# Autodesk Inventor assembly: WheelAssembly
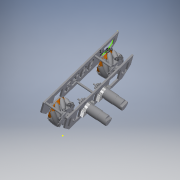
[picture p0: Inventor's stored thumbnail of the model, 180x180]
Saved by Autodesk Inventor 2017 (Build 210142000, 142)
## iProperties
Created: 2016-09-10
Part Number: WheelAssembly
Document SubType Name: Assembly
Designer: RoboticsUser
Author: RoboticsUser
## Documents named in this file (13)
- C:\Robotics\CAD\2016-17_CAD\Sub-Assemblies\MechanumNexus'AdaptorLeft - Copy.iam
- C:\Robotics\CAD\COTSParts\Actobotics\545 parts\545556.ipt
- C:\Robotics\CAD\COTSParts\Actobotics\615 parts\615102.ipt
- C:\Robotics\CAD\COTSParts\Actobotics\634 parts\634080.ipt
- C:\Robotics\CAD\COTSParts\Motors\Andymark 2964  NeveRest 40 Motor.ipt
- C:\Robotics\CAD\COTSParts\Tetrix\tetrix-motor-mounts-1.snapshot.1\Tetrex 2pc motor mount.ipt
- C:\Robotics\CAD\COTSParts\Actobotics\545 parts\545456.ipt
- C:\Robotics\CAD\COTSParts\Wheels\AndyMark Mecanum Wheels\100mm Aluminum Mecanum wheels.ipt
- C:\Robotics\CAD\2016-17_CAD\DriveTrain\DrainTrainPlate2.0LeftOutside.iam
- C:\Robotics\CAD\2016-17_CAD\DriveTrain\DriveTrainPlate2.0LeftInside.ipt
- C:\Robotics\CAD\COTSParts\Actobotics\535 parts\535198.ipt
- C:\Robotics\CAD\COTSParts\Actobotics\collar.ipt
- C:\Robotics\CAD\2016-17_CAD\DriveTrain\drive train standoff.ipt
## Components (35 placed, 12 different names)
1. 545556:2 — Mate:34, Mate:35, Mate:36, Mate:43
2. 615102:4 — Mate:62, Flush:6, Mate:65
3. 634080:2 — Mate:18, Flush:2, Mate:20, Mate:22, Mate:25, Mate:29, Mate:30, Mate:33, Mate:35, Mate:44, Mate:46, Mate:48
4. 545556:6 — Mate:8, Mate:17, Mate:27
5. 634080:3 — Mate:1, Mate:2, Mate:4, Mate:5, Mate:8, Mate:10, Mate:12, Flush:1, Mate:13, Mate:15, Mate:40, Mate:42, Mate:47
6. Andymark 2964  NeveRest 40 Motor:2 — Flush:3, Mate:59, Mate:62, Mate:66
7. 545556:8 — Mate:65, Mate:66
8. 545556:9 — Mate:63, Mate:64
9. Tetrex 2pc motor mount:1 — Mate:56, Mate:57, Mate:59
10. Tetrex 2pc motor mount:2 — Mate:58, Insert:1, Mate:60
11. 545456:1 — Mate:32, Mate:33, Mate:34, Mate:37
12. 545456:3 — Mate:9, Mate:10, Mate:27
13. 615102:6 — Flush:5, Mate:61, Mate:63
14. 615102:7 — Mate:36, Mate:37, Flush:5
15. 100mm Aluminum Mecanum wheels:1 — Mate:1, Mate:3, Mate:9
16. 100mm Aluminum Mecanum wheels:2 — Mate:30, Mate:31, Mate:32
17. 545456:4 — Mate:28, Mate:29, Mate:31
18. 545456:5 — Mate:2, Mate:3, Mate:7, Mate:38
19. 545556:13 — Mate:23, Mate:24, Mate:25, Mate:28
20. 545556:12 — Mate:4, Mate:38, Mate:39
21. DriveTrainPlate2.0LeftInside:1 — Mate:47, Mate:48, Mate:49, Mate:56, Mate:57, Mate:58, Insert:1, Flush:3, Flush:4
22. 615102:8 — Mate:5, Mate:7, Flush:6
23. 535198:2 — Mate:41, Mate:42
24. 535198:3 — Mate:45, Mate:46, Mate:49
25. 535198:4 — Mate:19, Mate:20, Mate:21
26. 535198:5 — Mate:14, Mate:15, Mate:16
27. collar:1 — Mate:21, Mate:22, Mate:23, Mate:24
28. collar:2 — Mate:13, Mate:16, Mate:17
29. Andymark 2964  NeveRest 40 Motor:3 — Flush:4, Mate:60, Mate:61, Mate:64
30. collar:3 — Mate:43, Mate:44, Mate:45
31. collar:4 — Mate:39, Mate:40, Mate:41
32. drive train standoff:1 — Mate:50, Mate:51
33. drive train standoff:2 — Mate:54, Mate:55
34. drive train standoff:3 — Mate:52, Mate:53
35. DrainTrainPlate2.0LeftOutside:1 [sub-assembly] — Mate:12, Flush:1, Mate:14, Mate:18, Flush:2, Mate:19, Mate:50, Mate:51, Mate:52, Mate:53, Mate:54, Mate:55
## Relationships (70: Mate 63, Flush 6, Insert 1)
- Mate:1: 634080:3 ↔ 100mm Aluminum Mecanum wheels:1
- Mate:2: 634080:3 ↔ 545456:5
- Mate:3: 100mm Aluminum Mecanum wheels:1 ↔ 545456:5
- Mate:4: 634080:3 ↔ 545556:12
- Mate:5: 634080:3 ↔ 615102:8
- Mate:7: 545456:5 ↔ 615102:8
- Mate:8: 545556:6 ↔ 634080:3
- Mate:9: 545456:3 ↔ 100mm Aluminum Mecanum wheels:1
- Mate:10: 634080:3 ↔ 545456:3
- Mate:12: 634080:3 ↔ DrainTrainPlate2.0LeftOutside:1
- Flush:1: 634080:3 ↔ DrainTrainPlate2.0LeftOutside:1
- Mate:13: 634080:3 ↔ collar:2
- Mate:14: 535198:5 ↔ DrainTrainPlate2.0LeftOutside:1
- Mate:15: 634080:3 ↔ 535198:5
- Mate:16: 535198:5 ↔ collar:2
- Mate:17: 545556:6 ↔ collar:2
- Mate:18: 634080:2 ↔ DrainTrainPlate2.0LeftOutside:1
- Flush:2: 634080:2 ↔ DrainTrainPlate2.0LeftOutside:1
- Mate:19: 535198:4 ↔ DrainTrainPlate2.0LeftOutside:1
- Mate:20: 634080:2 ↔ 535198:4
- Mate:21: 535198:4 ↔ collar:1
- Mate:22: 634080:2 ↔ collar:1
- Mate:23: 545556:13 ↔ collar:1
- Mate:24: 545556:13 ↔ collar:1
- Mate:25: 634080:2 ↔ 545556:13
- Mate:27: 545556:6 ↔ 545456:3
- Mate:28: 545456:4 ↔ 545556:13
- Mate:29: 634080:2 ↔ 545456:4
- Mate:30: 634080:2 ↔ 100mm Aluminum Mecanum wheels:2
- Mate:31: 100mm Aluminum Mecanum wheels:2 ↔ 545456:4
- Mate:32: 545456:1 ↔ 100mm Aluminum Mecanum wheels:2
- Mate:33: 634080:2 ↔ 545456:1
- Mate:34: 545556:2 ↔ 545456:1
- Mate:35: 545556:2 ↔ 634080:2
- Mate:36: 545556:2 ↔ 615102:7
- Mate:37: 545456:1 ↔ 615102:7
- Mate:38: 545456:5 ↔ 545556:12
- Mate:39: 545556:12 ↔ collar:4
- Mate:40: 634080:3 ↔ collar:4
- Mate:41: 535198:2 ↔ collar:4
- Mate:42: 634080:3 ↔ 535198:2
- Mate:43: 545556:2 ↔ collar:3
- Mate:44: 634080:2 ↔ collar:3
- Mate:45: 535198:3 ↔ collar:3
- Mate:46: 634080:2 ↔ 535198:3
- Mate:47: 634080:3 ↔ DriveTrainPlate2.0LeftInside:1
- Mate:48: 634080:2 ↔ DriveTrainPlate2.0LeftInside:1
- Mate:49: DriveTrainPlate2.0LeftInside:1 ↔ 535198:3
- Mate:50: drive train standoff:1 ↔ DrainTrainPlate2.0LeftOutside:1
- Mate:51: drive train standoff:1 ↔ DrainTrainPlate2.0LeftOutside:1
- Mate:52: drive train standoff:3 ↔ DrainTrainPlate2.0LeftOutside:1
- Mate:53: drive train standoff:3 ↔ DrainTrainPlate2.0LeftOutside:1
- Mate:54: drive train standoff:2 ↔ DrainTrainPlate2.0LeftOutside:1
- Mate:55: drive train standoff:2 ↔ DrainTrainPlate2.0LeftOutside:1
- Mate:56: Tetrex 2pc motor mount:1 ↔ DriveTrainPlate2.0LeftInside:1
- Mate:57: Tetrex 2pc motor mount:1 ↔ DriveTrainPlate2.0LeftInside:1
- Mate:58: Tetrex 2pc motor mount:2 ↔ DriveTrainPlate2.0LeftInside:1
- Insert:1: Tetrex 2pc motor mount:2 ↔ DriveTrainPlate2.0LeftInside:1
- Flush:3: Andymark 2964  NeveRest 40 Motor:2 ↔ DriveTrainPlate2.0LeftInside:1
- Mate:59: Andymark 2964  NeveRest 40 Motor:2 ↔ Tetrex 2pc motor mount:1
- Flush:4: DriveTrainPlate2.0LeftInside:1 ↔ Andymark 2964  NeveRest 40 Motor:3
- Mate:60: Tetrex 2pc motor mount:2 ↔ Andymark 2964  NeveRest 40 Motor:3
- Flush:5: 615102:6 ↔ 615102:7
- Mate:61: 615102:6 ↔ Andymark 2964  NeveRest 40 Motor:3
- Mate:62: 615102:4 ↔ Andymark 2964  NeveRest 40 Motor:2
- Flush:6: 615102:4 ↔ 615102:8
- Mate:63: 545556:9 ↔ 615102:6
- Mate:64: 545556:9 ↔ Andymark 2964  NeveRest 40 Motor:3
- Mate:65: 615102:4 ↔ 545556:8
- Mate:66: Andymark 2964  NeveRest 40 Motor:2 ↔ 545556:8
